# Autodesk Inventor assembly: assembly
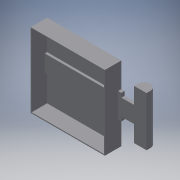
[picture p0: Inventor's stored thumbnail of the model, 180x180]
Saved by Autodesk Inventor 2017 (Build 210142000, 142)
## iProperties
Created: 2016-06-06
Part Number: assembly
Document SubType Name: Assembly
Designer: Conor
Author: Conor
## Documents named in this file (3)
- C:\Users\Conor\gravity_holder\assembly.iam
- C:\Users\Conor\gravity_holder\gravity_holder.ipt
- C:\Users\Conor\gravity_holder\weight_holder.ipt
## Components (2 placed, 2 different names)
1. gravity_holder:1 — Mate:1, Mate:2, Mate:3
2. weight_holder:1 — Mate:1, Mate:2, Mate:3
## Relationships (3: Mate 3)
- Mate:1: gravity_holder:1 ↔ weight_holder:1
- Mate:2: gravity_holder:1 ↔ weight_holder:1
- Mate:3: gravity_holder:1 ↔ weight_holder:1
